# Autodesk Inventor assembly: GreyT Telescope Gearbox_MIR
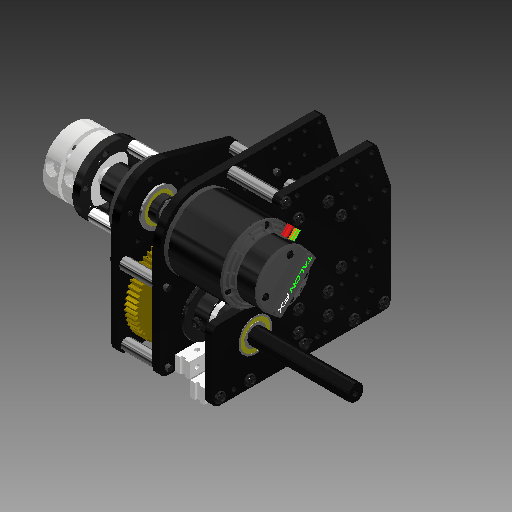
[picture p0: Inventor's stored thumbnail of the model, 512x512]
Saved by Autodesk Inventor 2022 (Build 260153000, 153)
## iProperties
Created: 2021-12-31
Part Number: GreyT Telescope Gearbox_MIR
Document SubType Name: Assembly
Revision Number: ANY
## Documents named in this file (39)
- C:\Users\Cal\Desktop\Robotics\Design\Collaborative\Collaborative Parts Library\Elevators\GreyT Telescope\GreyT Telescope Gearbox_MIR.iam
- C:\Users\Cal\Desktop\Robotics\Design\Collaborative\Collaborative Parts Library\Elevators\GreyT Telescope\WCP-0416-001 Rev1_MIR.ipt
- C:\Users\Cal\Desktop\Robotics\Design\Collaborative\Collaborative Parts Library\Elevators\GreyT Telescope\WCP-0416-002 Rev1_MIR.ipt
- C:\Users\Cal\Desktop\Robotics\Design\Collaborative\Collaborative Parts Library\Elevators\GreyT Telescope\WCP-0416-003 Rev1_MIR.ipt
- C:\Users\Cal\Desktop\Robotics\Design\Collaborative\Collaborative Parts Library\Elevators\GreyT Telescope\WCP-0225-006 Rev1.ipt
- C:\Users\Cal\Desktop\Robotics\Design\Collaborative\Collaborative Parts Library\Elevators\GreyT Telescope\WCP-0416-007 Rev1_1.5_ Gearbox.ipt
- C:\Users\Cal\Desktop\Robotics\Design\Collaborative\Collaborative Parts Library\Elevators\GreyT Telescope\WCP-0443 Rev1.ipt
- C:\Users\Cal\Desktop\Robotics\Design\Collaborative\Collaborative Parts Library\Motors\FRC\Falcon 500.ipt
- C:\Users\Cal\Desktop\Robotics\Design\Collaborative\Collaborative Parts Library\Elevators\GreyT Telescope\Falcon_Motor_Spacer_0625.ipt
- C:\Users\Cal\Desktop\Robotics\Design\Collaborative\Collaborative Parts Library\Power Transfer\Bearings and Bushings\Bearings\FR8.ipt
- C:\Users\Cal\Desktop\Robotics\Design\Collaborative\Collaborative Parts Library\Power Transfer\Bearings and Bushings\Bearings.ipt
- C:\Users\Cal\Desktop\Robotics\Design\Collaborative\Collaborative Parts Library\Power Transfer\Bearings and Bushings\Bearings\FR8 (Thunderhex).ipt
- C:\Users\Cal\Desktop\Robotics\Design\Collaborative\Collaborative Parts Library\Power Transfer\Bearings and Bushings\Bearings\FR8 Hex.ipt
- C:\Users\Cal\Desktop\Robotics\Design\Collaborative\Collaborative Parts Library\Power Transfer\Gears (Hex)\Spur Gear2\20dp 54T VexPro 500 Hex Aluminum Gear.ipt
- C:\Users\Cal\Desktop\Robotics\Design\Collaborative\Collaborative Parts Library\Power Transfer\Gears (Hex)\VexPro Spur Gears.ipt
- C:\Users\Cal\Desktop\Robotics\Design\Collaborative\Collaborative Parts Library\Power Transfer\Gears (Hex)\Spur Gear2\20dp 18T VexPro 500 Hex Steel Gear.ipt
- C:\Users\Cal\Desktop\Robotics\Design\Collaborative\Collaborative Parts Library\Hardware\Spacers\Spacers & Standoffs\WCP Aluminum Standoff (No. 10 x 1.125Lg x 0.375OD).ipt
- C:\Users\Cal\Desktop\Robotics\Design\Collaborative\Collaborative Parts Library\Hardware\Spacers\Spacers & Standoffs.ipt
- C:\Users\Cal\Desktop\Robotics\Design\Collaborative\Collaborative Parts Library\Hardware\Spacers\Spacers & Standoffs\WCP Aluminum Standoff (No. 10 x 1.5Lg x 0.375OD).ipt
- C:\Users\Cal\Desktop\Robotics\Design\Collaborative\Collaborative Parts Library\Hardware\Fasteners\Machine Screws\10-32 UNFx1.75 Button Head Cap Screw.ipt
- C:\Users\Cal\Desktop\Robotics\Design\Collaborative\Collaborative Parts Library\Hardware\Fasteners\Machine Screws.ipt
- C:\Users\Cal\Desktop\Robotics\Design\Collaborative\Collaborative Parts Library\Hardware\Fasteners\Machine Screws\10-32 UNFx0.5 Button Head Cap Screw.ipt
- C:\Users\Cal\Desktop\Robotics\Design\Collaborative\Collaborative Parts Library\Hardware\Fasteners\Machine Screws\10-32 UNFx0.375 Button Head Cap Screw.ipt
- C:\Users\Cal\Desktop\Robotics\Design\Collaborative\Collaborative Parts Library\Hardware\Fasteners\Machine Screws\10-32 UNFx2 Button Head Cap Screw.ipt
- C:\Users\Cal\Desktop\Robotics\Design\Collaborative\Collaborative Parts Library\Hardware\Spacers\Spacers & Standoffs\VexPro 500 Hex Spacer 0.25in.ipt
- C:\Users\Cal\Desktop\Robotics\Design\Collaborative\Collaborative Parts Library\Hardware\Spacers\Spacers & Standoffs\VexPro 500 Hex Spacer 0.0625in.ipt
- C:\Users\Cal\Desktop\Robotics\Design\Collaborative\Collaborative Parts Library\Roller Systems\VersaRoller End Cap.ipt
- C:\Users\Cal\Desktop\Robotics\Design\Collaborative\Collaborative Parts Library\Elevators\GreyT Telescope\217-3283 Rev1.ipt
- C:\Users\Cal\Desktop\Robotics\Design\Collaborative\Collaborative Parts Library\Elevators\GreyT Telescope\WCP-0282 Rev1.ipt
- C:\Users\Cal\Desktop\Robotics\Design\Collaborative\Collaborative Parts Library\Elevators\GreyT Telescope\WCP-0416-009 Rev1.ipt
- C:\Users\Cal\Desktop\Robotics\Design\Collaborative\Collaborative Parts Library\Shaft Retention\Snaprings\Snapring for 0.5in Shaft (0.461in).ipt
- C:\Users\Cal\Desktop\Robotics\Design\Collaborative\Collaborative Parts Library\Shaft Retention\Snaprings.ipt
- C:\Users\Cal\Desktop\Robotics\Design\Collaborative\Collaborative Parts Library\Elevators\GreyT Telescope\WCP-0229 Rev1.ipt
- C:\Users\Cal\Desktop\Robotics\Design\Collaborative\Collaborative Parts Library\Elevators\GreyT Telescope\WCP-0416-008 Rev1.ipt
- C:\Users\Cal\Desktop\Robotics\Design\Collaborative\Collaborative Parts Library\Elevators\GreyT Telescope\WCP-0416-010 Rev1.ipt
- C:\Users\Cal\Desktop\Robotics\Design\Collaborative\Collaborative Parts Library\Pneumatics\WCP-0200-Brake (500 Hex).iam
- C:\Users\Cal\Desktop\Robotics\Design\Collaborative\Collaborative Parts Library\Elevators\GreyT Telescope\CANcoder.ipt
- C:\Users\Cal\Desktop\Robotics\Design\Collaborative\Collaborative Parts Library\Elevators\GreyT Telescope\WCP-0156 Rev1.ipt
- C:\Users\Cal\Desktop\Robotics\Design\Collaborative\Collaborative Parts Library\Power Transfer\Motor Output\Gears\Falcon 8T Pinion (VexPro #217-6915).ipt
## Components (78 placed, 33 different names)
1. WCP-0416-001 Rev1_MIR:1 — Insert:57, Insert:58, Mate:1, Insert:1, Insert:20, Insert:21, Insert:8, Insert:14, Insert:9, Insert:15, Insert:35, Insert:33, Insert:34, Insert:39, Insert:38, Insert:36, Insert:37, Insert:45, Insert:44, Insert:51
2. WCP-0416-002 Rev1_MIR:1 — Angle:1, Insert:54, Mate:6, Insert:55, Insert:2, Insert:3, Insert:4, Insert:5, Insert:43, Insert:41, Insert:40, Insert:42, Insert:48, Insert:50, Insert:53
3. WCP-0416-003 Rev1_MIR:1 — Insert:56, Insert:59, Insert:11, Insert:12, Insert:10, Insert:13, Insert:19, Insert:18, Insert:16, Insert:17, Insert:26, Insert:29, Insert:31, Insert:30, Insert:27, Insert:28, Insert:32, Insert:46, Insert:47, Insert:52
4. WCP-0225-006 Rev1:1 — Insert:49
5. WCP-0416-007 Rev1_1.5_ Gearbox:1 — Insert:64, Insert:63, Mate:9, Mate:7, Mate:10, Mate:8
6. WCP-0443 Rev1:1 — Insert:64
7. WCP-0443 Rev1:2 — Insert:63
8. Falcon 500:1 — Mate:1, Insert:1, Insert:73
9. Falcon_Motor_Spacer_0625:1 — Insert:74
10. FR8:1 — Insert:49, Insert:48
11. FR8:2 — Insert:51, Insert:60
12. FR8 (Thunderhex):3 — Insert:52, Insert:65
13. FR8 Hex:4 — Insert:53, Insert:67
14. FR8:5 — Insert:69, Insert:50, Insert:61, Insert:66
15. 20dp 54T VexPro 500 Hex Aluminum Gear:1 — Insert:60, Insert:62
16. 20dp 54T VexPro 500 Hex Aluminum Gear:2 — Insert:61
17. 20dp 18T VexPro 500 Hex Steel Gear:3 — Insert:62
18. WCP Aluminum Standoff (No. 10 x 1.125Lg x 0.375OD):1 — Insert:45, Insert:43
19. WCP Aluminum Standoff (No. 10 x 1.125Lg x 0.375OD):2 — Insert:41
20. WCP Aluminum Standoff (No. 10 x 1.5Lg x 0.375OD):3 — Insert:35
21. WCP Aluminum Standoff (No. 10 x 1.5Lg x 0.375OD):4 — Insert:46, Insert:33
22. WCP Aluminum Standoff (No. 10 x 1.5Lg x 0.375OD):5 — Insert:47, Insert:34
23. WCP Aluminum Standoff (No. 10 x 1.5Lg x 0.375OD):6 — Insert:39
24. WCP Aluminum Standoff (No. 10 x 1.5Lg x 0.375OD):7 — Insert:38
25. WCP Aluminum Standoff (No. 10 x 1.5Lg x 0.375OD):8 — Insert:36
26. WCP Aluminum Standoff (No. 10 x 1.125Lg x 0.375OD):9 — Insert:40
27. WCP Aluminum Standoff (No. 10 x 1.125Lg x 0.375OD):10 — Insert:44, Insert:42
28. WCP Aluminum Standoff (No. 10 x 1.5Lg x 0.375OD):11 — Insert:37
29. 10-32 UNFx1.75 Button Head Cap Screw:1 — Insert:2
30. 10-32 UNFx1.75 Button Head Cap Screw:2 — Insert:3
31. 10-32 UNFx1.75 Button Head Cap Screw:3 — Insert:4
32. 10-32 UNFx1.75 Button Head Cap Screw:4 — Insert:5
33. 10-32 UNFx0.5 Button Head Cap Screw:5 — Insert:6
34. 10-32 UNFx0.5 Button Head Cap Screw:6 — Insert:7
35. 10-32 UNFx0.375 Button Head Cap Screw:7 — Insert:19
36. 10-32 UNFx0.375 Button Head Cap Screw:8 — Insert:18
37. 10-32 UNFx0.375 Button Head Cap Screw:9 — Insert:16
38. 10-32 UNFx0.375 Button Head Cap Screw:10 — Insert:17
39. 10-32 UNFx2 Button Head Cap Screw:11 — Insert:26
40. 10-32 UNFx2 Button Head Cap Screw:12 — Insert:29
41. 10-32 UNFx2 Button Head Cap Screw:13 — Insert:31
42. 10-32 UNFx2 Button Head Cap Screw:14 — Insert:30
43. 10-32 UNFx2 Button Head Cap Screw:15 — Insert:27
44. 10-32 UNFx2 Button Head Cap Screw:16 — Insert:28
45. 10-32 UNFx0.5 Button Head Cap Screw:17 — Insert:20
46. 10-32 UNFx0.5 Button Head Cap Screw:18 — Insert:21
47. 10-32 UNFx0.5 Button Head Cap Screw:19 — Insert:8
48. 10-32 UNFx0.5 Button Head Cap Screw:20 — Insert:14
49. 10-32 UNFx0.5 Button Head Cap Screw:21 — Insert:9
50. 10-32 UNFx0.5 Button Head Cap Screw:22 — Insert:11
51. 10-32 UNFx0.5 Button Head Cap Screw:23 — Insert:12
52. 10-32 UNFx0.5 Button Head Cap Screw:24 — Insert:10
53. 10-32 UNFx0.5 Button Head Cap Screw:25 — Insert:13
54. 10-32 UNFx0.5 Button Head Cap Screw:26 — Insert:15
55. 10-32 UNFx2 Button Head Cap Screw:27 — Insert:32
56. VexPro 500 Hex Spacer 0.25in:12 — Insert:72, Insert:67
57. VexPro 500 Hex Spacer 0.0625in:13 — Insert:65
58. VexPro 500 Hex Spacer 0.0625in:14 — Insert:66
59. VersaRoller End Cap:1 — Mate:9, Mate:7
60. 217-3283 Rev1:1 — Insert:68, Insert:69, Insert:70
61. WCP-0282 Rev1:1 — Insert:71
62. WCP-0416-009 Rev1:1 — Insert:56, Flush:1
63. WCP-0416-009 Rev1:2 — Flush:1, Insert:57
64. WCP-0416-009 Rev1:3 — Insert:59, Flush:2
65. WCP-0416-009 Rev1:4 — Flush:2, Insert:58
66. Snapring for 0.5in Shaft (0.461in):1 — Insert:70
67. WCP-0229 Rev1:1 — Insert:71, Insert:72
68. WCP-0416-008 Rev1:1 — Angle:1, Insert:54, Mate:5, Mate:4, Mate:3, Insert:6, Insert:7
69. WCP-0416-010 Rev1:1 — Insert:75
70. WCP-0200-Brake (500 Hex):1 [sub-assembly] — Mate:6, Insert:55, Insert:22, Insert:23, Insert:24, Insert:25
71. 10-32 UNFx0.5 Button Head Cap Screw:28 — Insert:22
72. 10-32 UNFx0.5 Button Head Cap Screw:29 — Insert:23
73. 10-32 UNFx0.5 Button Head Cap Screw:30 — Insert:24
74. 10-32 UNFx0.5 Button Head Cap Screw:31 — Insert:25
75. CANcoder:1 — Mate:5, Mate:4, Mate:3
76. WCP-0156 Rev1:1 — Insert:68
77. Falcon 8T Pinion (VexPro #217-6915):1 — Insert:74, Insert:73
78. VersaRoller End Cap:2 — Insert:75, Mate:10, Mate:8
## Relationships (87: Insert 75, Mate 9, Flush 2, Angle 1)
- Insert:64: WCP-0416-007 Rev1_1.5_ Gearbox:1 ↔ WCP-0443 Rev1:1
- Insert:63: WCP-0416-007 Rev1_1.5_ Gearbox:1 ↔ WCP-0443 Rev1:2
- Insert:56: WCP-0416-003 Rev1_MIR:1 ↔ WCP-0416-009 Rev1:1
- Flush:1: WCP-0416-009 Rev1:1 ↔ WCP-0416-009 Rev1:2
- Insert:57: WCP-0416-001 Rev1_MIR:1 ↔ WCP-0416-009 Rev1:2
- Insert:59: WCP-0416-003 Rev1_MIR:1 ↔ WCP-0416-009 Rev1:3
- Flush:2: WCP-0416-009 Rev1:3 ↔ WCP-0416-009 Rev1:4
- Insert:58: WCP-0416-001 Rev1_MIR:1 ↔ WCP-0416-009 Rev1:4
- Insert:71: WCP-0282 Rev1:1 ↔ WCP-0229 Rev1:1
- Angle:1 (0 deg): WCP-0416-002 Rev1_MIR:1 ↔ WCP-0416-008 Rev1:1
- Insert:54: WCP-0416-002 Rev1_MIR:1 ↔ WCP-0416-008 Rev1:1
- Mate:5: WCP-0416-008 Rev1:1 ↔ CANcoder:1
- Mate:4: WCP-0416-008 Rev1:1 ↔ CANcoder:1
- Mate:3: WCP-0416-008 Rev1:1 ↔ CANcoder:1
- Insert:68: 217-3283 Rev1:1 ↔ WCP-0156 Rev1:1
- Mate:6: WCP-0416-002 Rev1_MIR:1 ↔ WCP-0200-Brake (500 Hex):1
- Insert:55: WCP-0416-002 Rev1_MIR:1 ↔ WCP-0200-Brake (500 Hex):1
- Mate:1: WCP-0416-001 Rev1_MIR:1 ↔ Falcon 500:1
- Insert:1: WCP-0416-001 Rev1_MIR:1 ↔ Falcon 500:1
- Insert:2: WCP-0416-002 Rev1_MIR:1 ↔ 10-32 UNFx1.75 Button Head Cap Screw:1
- Insert:3: WCP-0416-002 Rev1_MIR:1 ↔ 10-32 UNFx1.75 Button Head Cap Screw:2
- Insert:4: WCP-0416-002 Rev1_MIR:1 ↔ 10-32 UNFx1.75 Button Head Cap Screw:3
- Insert:5: WCP-0416-002 Rev1_MIR:1 ↔ 10-32 UNFx1.75 Button Head Cap Screw:4
- Insert:6: 10-32 UNFx0.5 Button Head Cap Screw:5 ↔ WCP-0416-008 Rev1:1
- Insert:7: 10-32 UNFx0.5 Button Head Cap Screw:6 ↔ WCP-0416-008 Rev1:1
- Insert:20: WCP-0416-001 Rev1_MIR:1 ↔ 10-32 UNFx0.5 Button Head Cap Screw:17
- Insert:21: WCP-0416-001 Rev1_MIR:1 ↔ 10-32 UNFx0.5 Button Head Cap Screw:18
- Insert:8: WCP-0416-001 Rev1_MIR:1 ↔ 10-32 UNFx0.5 Button Head Cap Screw:19
- Insert:14: WCP-0416-001 Rev1_MIR:1 ↔ 10-32 UNFx0.5 Button Head Cap Screw:20
- Insert:9: WCP-0416-001 Rev1_MIR:1 ↔ 10-32 UNFx0.5 Button Head Cap Screw:21
- Insert:11: WCP-0416-003 Rev1_MIR:1 ↔ 10-32 UNFx0.5 Button Head Cap Screw:22
- Insert:12: WCP-0416-003 Rev1_MIR:1 ↔ 10-32 UNFx0.5 Button Head Cap Screw:23
- Insert:10: WCP-0416-003 Rev1_MIR:1 ↔ 10-32 UNFx0.5 Button Head Cap Screw:24
- Insert:13: WCP-0416-003 Rev1_MIR:1 ↔ 10-32 UNFx0.5 Button Head Cap Screw:25
- Insert:15: WCP-0416-001 Rev1_MIR:1 ↔ 10-32 UNFx0.5 Button Head Cap Screw:26
- Insert:22: WCP-0200-Brake (500 Hex):1 ↔ 10-32 UNFx0.5 Button Head Cap Screw:28
- Insert:23: WCP-0200-Brake (500 Hex):1 ↔ 10-32 UNFx0.5 Button Head Cap Screw:29
- Insert:24: WCP-0200-Brake (500 Hex):1 ↔ 10-32 UNFx0.5 Button Head Cap Screw:30
- Insert:25: WCP-0200-Brake (500 Hex):1 ↔ 10-32 UNFx0.5 Button Head Cap Screw:31
- Insert:19: WCP-0416-003 Rev1_MIR:1 ↔ 10-32 UNFx0.375 Button Head Cap Screw:7
- Insert:18: WCP-0416-003 Rev1_MIR:1 ↔ 10-32 UNFx0.375 Button Head Cap Screw:8
- Insert:16: WCP-0416-003 Rev1_MIR:1 ↔ 10-32 UNFx0.375 Button Head Cap Screw:9
- Insert:17: WCP-0416-003 Rev1_MIR:1 ↔ 10-32 UNFx0.375 Button Head Cap Screw:10
- Insert:26: WCP-0416-003 Rev1_MIR:1 ↔ 10-32 UNFx2 Button Head Cap Screw:11
- Insert:29: WCP-0416-003 Rev1_MIR:1 ↔ 10-32 UNFx2 Button Head Cap Screw:12
- Insert:31: WCP-0416-003 Rev1_MIR:1 ↔ 10-32 UNFx2 Button Head Cap Screw:13
- Insert:30: WCP-0416-003 Rev1_MIR:1 ↔ 10-32 UNFx2 Button Head Cap Screw:14
- Insert:27: WCP-0416-003 Rev1_MIR:1 ↔ 10-32 UNFx2 Button Head Cap Screw:15
- Insert:28: WCP-0416-003 Rev1_MIR:1 ↔ 10-32 UNFx2 Button Head Cap Screw:16
- Insert:32: WCP-0416-003 Rev1_MIR:1 ↔ 10-32 UNFx2 Button Head Cap Screw:27
- Insert:35: WCP-0416-001 Rev1_MIR:1 ↔ WCP Aluminum Standoff (No. 10 x 1.5Lg x 0.375OD):3
- Insert:46: WCP-0416-003 Rev1_MIR:1 ↔ WCP Aluminum Standoff (No. 10 x 1.5Lg x 0.375OD):4
- Insert:33: WCP-0416-001 Rev1_MIR:1 ↔ WCP Aluminum Standoff (No. 10 x 1.5Lg x 0.375OD):4
- Insert:47: WCP-0416-003 Rev1_MIR:1 ↔ WCP Aluminum Standoff (No. 10 x 1.5Lg x 0.375OD):5
- Insert:34: WCP-0416-001 Rev1_MIR:1 ↔ WCP Aluminum Standoff (No. 10 x 1.5Lg x 0.375OD):5
- Insert:39: WCP-0416-001 Rev1_MIR:1 ↔ WCP Aluminum Standoff (No. 10 x 1.5Lg x 0.375OD):6
- Insert:38: WCP-0416-001 Rev1_MIR:1 ↔ WCP Aluminum Standoff (No. 10 x 1.5Lg x 0.375OD):7
- Insert:36: WCP-0416-001 Rev1_MIR:1 ↔ WCP Aluminum Standoff (No. 10 x 1.5Lg x 0.375OD):8
- Insert:37: WCP-0416-001 Rev1_MIR:1 ↔ WCP Aluminum Standoff (No. 10 x 1.5Lg x 0.375OD):11
- Insert:45: WCP-0416-001 Rev1_MIR:1 ↔ WCP Aluminum Standoff (No. 10 x 1.125Lg x 0.375OD):1
- Insert:43: WCP-0416-002 Rev1_MIR:1 ↔ WCP Aluminum Standoff (No. 10 x 1.125Lg x 0.375OD):1
- Insert:41: WCP-0416-002 Rev1_MIR:1 ↔ WCP Aluminum Standoff (No. 10 x 1.125Lg x 0.375OD):2
- Insert:40: WCP-0416-002 Rev1_MIR:1 ↔ WCP Aluminum Standoff (No. 10 x 1.125Lg x 0.375OD):9
- Insert:44: WCP-0416-001 Rev1_MIR:1 ↔ WCP Aluminum Standoff (No. 10 x 1.125Lg x 0.375OD):10
- Insert:42: WCP-0416-002 Rev1_MIR:1 ↔ WCP Aluminum Standoff (No. 10 x 1.125Lg x 0.375OD):10
- Insert:49: WCP-0225-006 Rev1:1 ↔ FR8:1
- Insert:48: WCP-0416-002 Rev1_MIR:1 ↔ FR8:1
- Insert:51: WCP-0416-001 Rev1_MIR:1 ↔ FR8:2
- Insert:69: FR8:5 ↔ 217-3283 Rev1:1
- Insert:50: WCP-0416-002 Rev1_MIR:1 ↔ FR8:5
- Insert:52: WCP-0416-003 Rev1_MIR:1 ↔ FR8 (Thunderhex):3
- Insert:53: WCP-0416-002 Rev1_MIR:1 ↔ FR8 Hex:4
- Insert:60: FR8:2 ↔ 20dp 54T VexPro 500 Hex Aluminum Gear:1
- Insert:61 (1.5875 mm): FR8:5 ↔ 20dp 54T VexPro 500 Hex Aluminum Gear:2
- Insert:62: 20dp 54T VexPro 500 Hex Aluminum Gear:1 ↔ 20dp 18T VexPro 500 Hex Steel Gear:3
- Insert:65: FR8 (Thunderhex):3 ↔ VexPro 500 Hex Spacer 0.0625in:13
- Insert:66: FR8:5 ↔ VexPro 500 Hex Spacer 0.0625in:14
- Insert:72: VexPro 500 Hex Spacer 0.25in:12 ↔ WCP-0229 Rev1:1
- Insert:67: FR8 Hex:4 ↔ VexPro 500 Hex Spacer 0.25in:12
- Insert:70: 217-3283 Rev1:1 ↔ Snapring for 0.5in Shaft (0.461in):1
- Insert:74: Falcon_Motor_Spacer_0625:1 ↔ Falcon 8T Pinion (VexPro #217-6915):1
- Insert:73: Falcon 500:1 ↔ Falcon 8T Pinion (VexPro #217-6915):1
- Mate:9: WCP-0416-007 Rev1_1.5_ Gearbox:1 ↔ VersaRoller End Cap:1
- Mate:7: WCP-0416-007 Rev1_1.5_ Gearbox:1 ↔ VersaRoller End Cap:1
- Insert:75: WCP-0416-010 Rev1:1 ↔ VersaRoller End Cap:2
- Mate:10: WCP-0416-007 Rev1_1.5_ Gearbox:1 ↔ VersaRoller End Cap:2
- Mate:8: WCP-0416-007 Rev1_1.5_ Gearbox:1 ↔ VersaRoller End Cap:2
